# Autodesk Inventor assembly: Manipulator
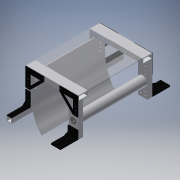
[picture p0: Inventor's stored thumbnail of the model, 180x180]
Saved by Autodesk Inventor 2016 (Build 200138000, 138)
## iProperties
Created: 2016-01-16
Part Number: Manipulator
Description: STEP AP214
Document SubType Name: Assembly
Designer: Douglas
Sending System: SolidWorks 2015
Preprocessor: SwSTEP 2.0
Title: Manipulator.STEP
Revision Number: ANY
## Documents named in this file (13)
- D:\SkyDrive\GitHub\2016-Robot-CAD\Inventor\PARTS\Manipulator\Manipulator.iam
- D:\SkyDrive\GitHub\2016-Robot-CAD\Inventor\PARTS\Lift\Side Support Beam 23.5 in.ipt
- D:\SkyDrive\GitHub\2016-Robot-CAD\Inventor\PARTS\Lift\Manipulator Motor Support.ipt
- D:\SkyDrive\GitHub\2016-Robot-CAD\Inventor\PARTS\Lift\Spinner.ipt
- D:\SkyDrive\GitHub\2016-Robot-CAD\Inventor\PARTS\Lift\Ramp.ipt
- D:\SkyDrive\GitHub\2016-Robot-CAD\Inventor\PARTS\Lift\1-8 Bar Back of Ramp.ipt
- D:\SkyDrive\GitHub\2016-Robot-CAD\Inventor\PARTS\Lift\1-8 in top plate for ramp.ipt
- D:\SkyDrive\GitHub\2016-Robot-CAD\Inventor\PARTS\Lift\Top Support Manipulator.ipt
- D:\SkyDrive\GitHub\2016-Robot-CAD\Inventor\PARTS\Lift\L Bracket 1.ipt
- D:\SkyDrive\GitHub\2016-Robot-CAD\Inventor\PARTS\Lift\L Bracket 2.ipt
- D:\SkyDrive\GitHub\2016-Robot-CAD\Inventor\PARTS\Lift\L Bracket 3.ipt
- D:\SkyDrive\GitHub\2016-Robot-CAD\Inventor\PARTS\Lift\L Bracket Front Manipulator.ipt
- D:\SkyDrive\GitHub\2016-Robot-CAD\Inventor\PARTS\Lift\FR8ZZ Hex Bearing.ipt
## Components (24 placed, 24 different names)
1. Side Support Beam 23.5 in_1 — Mate:1, Mate:2, Mate:3, Mate:4, Mate:5, Mate:6, Mate:7, Mate:10, Mate:16, Mate:19
2. Manipulator Motor Support_2 — Mate:47, Flush:9, Mate:48, Mate:49, Mate:50, Flush:10, Mate:55
3. Manipulator Motor Support_3 — Mate:38, Mate:39, Flush:8, Mate:40, Mate:41, Mate:44, Mate:45, Mate:46, Mate:51, Mate:52
4. Spinner_4 — Mate:42, Mate:43
5. Ramp_5 — Mate:13, Mate:14, Flush:5
6. 1-8 Bar Back of Ramp_6 — Mate:7, Mate:8, Mate:9, Mate:13, Mate:14, Flush:2, Mate:20, Mate:21, Mate:25, Mate:28, Mate:31
7. 1-8 Bar Back of Ramp_7 — Mate:10, Mate:11, Mate:12, Flush:3, Mate:17, Mate:18, Mate:34, Mate:58
8. 1-8 in top plate for ramp_8 — Flush:2, Flush:3, Mate:22, Flush:4, Mate:24, Flush:6, Flush:7
9. Top Support Manipulator_9 — Mate:24, Flush:5, Flush:7, Mate:25, Mate:26, Mate:27, Mate:29, Mate:30, Mate:35, Mate:36, Mate:37, Mate:38, Flush:8
10. Top Support Manipulator_10 — Mate:22, Flush:4, Flush:6, Mate:32, Mate:33, Mate:47, Flush:9, Flush:10, Mate:53, Mate:54, Mate:56, Mate:57
11. L Bracket 1_11 — Mate:56, Mate:57, Mate:58
12. L Bracket 1_12 — Mate:53, Mate:54, Mate:55
13. L Bracket 1_13 — Mate:26, Mate:27, Mate:28
14. L Bracket 1_14 — Mate:35, Mate:36, Mate:37, Mate:39
15. L Bracket 2_15 — Mate:32, Mate:33, Mate:34
16. L Bracket 2_16 — Mate:29, Mate:30, Mate:31
17. L Bracket 3_17 — Mate:4, Mate:5, Mate:6, Mate:11, Mate:12
18. L Bracket 3_18 — Mate:16, Mate:17, Mate:18
19. L Bracket 3_19 — Mate:19, Mate:20, Mate:21
20. L Bracket 3_20 — Mate:1, Mate:2, Mate:3, Mate:8, Mate:9
21. L Bracket Front Manipulator_21 — Mate:48, Mate:49, Mate:50
22. L Bracket Front Manipulator_22 — Mate:44, Mate:45, Mate:46
23. FR8ZZ Hex Bearing_23 — Mate:51, Mate:52
24. FR8ZZ Hex Bearing_24 — Mate:40, Mate:41, Mate:42, Mate:43
## Relationships (65: Mate 56, Flush 9)
- Mate:1: Side Support Beam 23.5 in_1 ↔ L Bracket 3_20
- Mate:2: Side Support Beam 23.5 in_1 ↔ L Bracket 3_20
- Mate:3: Side Support Beam 23.5 in_1 ↔ L Bracket 3_20
- Mate:4: Side Support Beam 23.5 in_1 ↔ L Bracket 3_17
- Mate:5: Side Support Beam 23.5 in_1 ↔ L Bracket 3_17
- Mate:6: Side Support Beam 23.5 in_1 ↔ L Bracket 3_17
- Mate:7: Side Support Beam 23.5 in_1 ↔ 1-8 Bar Back of Ramp_6
- Mate:8: 1-8 Bar Back of Ramp_6 ↔ L Bracket 3_20
- Mate:9: 1-8 Bar Back of Ramp_6 ↔ L Bracket 3_20
- Mate:10: Side Support Beam 23.5 in_1 ↔ 1-8 Bar Back of Ramp_7
- Mate:11: 1-8 Bar Back of Ramp_7 ↔ L Bracket 3_17
- Mate:12: 1-8 Bar Back of Ramp_7 ↔ L Bracket 3_17
- Mate:13: Ramp_5 ↔ 1-8 Bar Back of Ramp_6
- Mate:14: Ramp_5 ↔ 1-8 Bar Back of Ramp_6
- Flush:2: 1-8 Bar Back of Ramp_6 ↔ 1-8 in top plate for ramp_8
- Flush:3: 1-8 Bar Back of Ramp_7 ↔ 1-8 in top plate for ramp_8
- Mate:16: Side Support Beam 23.5 in_1 ↔ L Bracket 3_18
- Mate:17: 1-8 Bar Back of Ramp_7 ↔ L Bracket 3_18
- Mate:18: 1-8 Bar Back of Ramp_7 ↔ L Bracket 3_18
- Mate:19: Side Support Beam 23.5 in_1 ↔ L Bracket 3_19
- Mate:20: 1-8 Bar Back of Ramp_6 ↔ L Bracket 3_19
- Mate:21: 1-8 Bar Back of Ramp_6 ↔ L Bracket 3_19
- Mate:22: 1-8 in top plate for ramp_8 ↔ Top Support Manipulator_10
- Flush:4: 1-8 in top plate for ramp_8 ↔ Top Support Manipulator_10
- Mate:24: 1-8 in top plate for ramp_8 ↔ Top Support Manipulator_9
- Flush:5: Ramp_5 ↔ Top Support Manipulator_9
- Flush:6: 1-8 in top plate for ramp_8 ↔ Top Support Manipulator_10
- Flush:7: 1-8 in top plate for ramp_8 ↔ Top Support Manipulator_9
- Mate:25: 1-8 Bar Back of Ramp_6 ↔ Top Support Manipulator_9
- Mate:26: Top Support Manipulator_9 ↔ L Bracket 1_13
- Mate:27: Top Support Manipulator_9 ↔ L Bracket 1_13
- Mate:28: 1-8 Bar Back of Ramp_6 ↔ L Bracket 1_13
- Mate:29: Top Support Manipulator_9 ↔ L Bracket 2_16
- Mate:30: Top Support Manipulator_9 ↔ L Bracket 2_16
- Mate:31: 1-8 Bar Back of Ramp_6 ↔ L Bracket 2_16
- Mate:32: Top Support Manipulator_10 ↔ L Bracket 2_15
- Mate:33: Top Support Manipulator_10 ↔ L Bracket 2_15
- Mate:34: 1-8 Bar Back of Ramp_7 ↔ L Bracket 2_15
- Mate:35: Top Support Manipulator_9 ↔ L Bracket 1_14
- Mate:36: Top Support Manipulator_9 ↔ L Bracket 1_14
- Mate:37: Top Support Manipulator_9 ↔ L Bracket 1_14
- Mate:38: Manipulator Motor Support_3 ↔ Top Support Manipulator_9
- Mate:39: Manipulator Motor Support_3 ↔ L Bracket 1_14
- Flush:8: Manipulator Motor Support_3 ↔ Top Support Manipulator_9
- Mate:40: Manipulator Motor Support_3 ↔ FR8ZZ Hex Bearing_24
- Mate:41: Manipulator Motor Support_3 ↔ FR8ZZ Hex Bearing_24
- Mate:42: Spinner_4 ↔ FR8ZZ Hex Bearing_24
- Mate:43: Spinner_4 ↔ FR8ZZ Hex Bearing_24
- Mate:44: Manipulator Motor Support_3 ↔ L Bracket Front Manipulator_22
- Mate:45: Manipulator Motor Support_3 ↔ L Bracket Front Manipulator_22
- Mate:46: Manipulator Motor Support_3 ↔ L Bracket Front Manipulator_22
- Mate:47: Manipulator Motor Support_2 ↔ Top Support Manipulator_10
- Flush:9: Manipulator Motor Support_2 ↔ Top Support Manipulator_10
- Mate:48: Manipulator Motor Support_2 ↔ L Bracket Front Manipulator_21
- Mate:49: Manipulator Motor Support_2 ↔ L Bracket Front Manipulator_21
- Mate:50: Manipulator Motor Support_2 ↔ L Bracket Front Manipulator_21
- Mate:51: Manipulator Motor Support_3 ↔ FR8ZZ Hex Bearing_23
- Mate:52: Manipulator Motor Support_3 ↔ FR8ZZ Hex Bearing_23
- Flush:10: Manipulator Motor Support_2 ↔ Top Support Manipulator_10
- Mate:53: Top Support Manipulator_10 ↔ L Bracket 1_12
- Mate:54: Top Support Manipulator_10 ↔ L Bracket 1_12
- Mate:55: Manipulator Motor Support_2 ↔ L Bracket 1_12
- Mate:56: Top Support Manipulator_10 ↔ L Bracket 1_11
- Mate:57: Top Support Manipulator_10 ↔ L Bracket 1_11
- Mate:58: 1-8 Bar Back of Ramp_7 ↔ L Bracket 1_11
